# Autodesk Inventor assembly: RF603_stativ
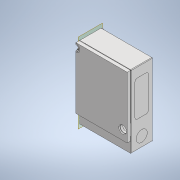
[picture p0: Inventor's stored thumbnail of the model, 180x180]
Saved by Autodesk Inventor 2022 (Build 260153000, 153)
## iProperties
Created: 2022-01-02
Part Number: RF603_stativ
Document SubType Name: Assembly
Designer: Jan
Author: Jan
## Documents named in this file (5)
- C:\Users\Jan\Documents\RF603_stativ.iam
- C:\Users\Jan\Desktop\RF603_DEMO\RF603RF603_2CC.iam
- C:\Users\Jan\Documents\stativ.ipt
- C:\Users\Jan\Documents\Hülse1.ipt
- C:\Users\Jan\Documents\Hülse2.ipt
## Components (4 placed, 4 different names)
1. RF603RF603_2CC:1 [sub-assembly] — Fluchtend:1, Winkel:1
2. stativ:1 — Fluchtend:1
3. Hülse1:1 — Fluchtend:2
4. Hülse2:1 — Fluchtend:3
## Relationships (4: Flush 3, Angle 1)
- Fluchtend:1 [Flush]: RF603RF603_2CC:1 ↔ stativ:1
- Winkel:1 [Angle] (0 deg): RF603RF603_2CC:1
- Fluchtend:2 [Flush]: Hülse1:1
- Fluchtend:3 [Flush]: Hülse2:1
